# Autodesk Inventor assembly: example_casing+servo
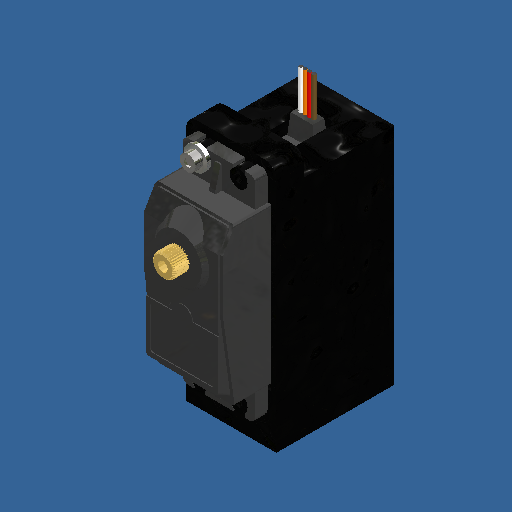
[picture p0: Inventor's stored thumbnail of the model, 512x512]
Saved by Autodesk Inventor 2026.2 (Build 302298000, 298)
## iProperties
Created: 2026-01-15
Part Number: example_casing+servo
Document SubType Name: Assembly
Designer: Thoma
Author: Thoma
## Documents named in this file (5)
- C:\Users\Thoma\OneDrive\Desktop\dir\telescope_cover\cover\example_casing+servo.iam
- C:\Users\Thoma\OneDrive\Desktop\dir\telescope_cover\servo\DSS-M15S Servo.ipt
- C:\Users\Thoma\OneDrive\Desktop\dir\telescope_cover\cover\casing_v2.ipt
- C:\Users\Thoma\OneDrive\Desktop\dir\telescope_cover\cover\8mm_washer_1mm.ipt
- C:\Users\Thoma\OneDrive\Desktop\dir\telescope_cover\cover\4mm_screw.ipt
## Components (4 placed, 4 different names)
1. DSS-M15S Servo:1 — Mate:3, Mate:6, Mate:7
2. casing_v2:1 — Mate:3, Mate:4, Mate:5, Mate:6, Mate:7, Mate:8, Angle:1
3. 8mm_washer_1mm:1 — Mate:4, Mate:5, Mate:9
4. 4mm_screw:1 — Mate:8, Mate:9, Angle:1
## Relationships (8: Mate 7, Angle 1)
- Mate:3: DSS-M15S Servo:1 ↔ casing_v2:1
- Mate:4: casing_v2:1 ↔ 8mm_washer_1mm:1
- Mate:5: casing_v2:1 ↔ 8mm_washer_1mm:1
- Mate:6 (0.1 mm): DSS-M15S Servo:1 ↔ casing_v2:1
- Mate:7 (0.1 mm): DSS-M15S Servo:1 ↔ casing_v2:1
- Mate:8: casing_v2:1 ↔ 4mm_screw:1
- Mate:9: 8mm_washer_1mm:1 ↔ 4mm_screw:1
- Angle:1 (0 deg): casing_v2:1 ↔ 4mm_screw:1
